# Autodesk Inventor assembly: ManualClamp
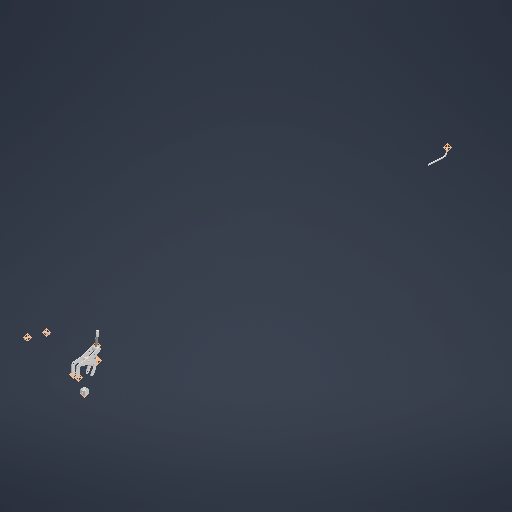
[picture p0: Inventor's stored thumbnail of the model, 512x512]
Saved by Autodesk Inventor 2025.4 (Build 294407000, 407)
## iProperties
Created: 2026-05-27
Part Number: ManualClamp
Document SubType Name: Assembly
Designer: VuQuan
Author: VuQuan
## Documents named in this file (12)
- D:\Edu\4CHaUI-Inventor\Assambly\b1\clamp\ManualClamp.iam
- D:\Edu\4CHaUI-Inventor\Assambly\b1\clamp\Base.ipt
- D:\Edu\4CHaUI-Inventor\Assambly\b1\clamp\BaseSpacer.ipt
- D:\Edu\4CHaUI-Inventor\Assambly\b1\clamp\BaseSupport.ipt
- D:\Edu\4CHaUI-Inventor\Assambly\b1\clamp\Elbow.ipt
- D:\Edu\4CHaUI-Inventor\Assambly\b1\clamp\Foot.ipt
- D:\Edu\4CHaUI-Inventor\Assambly\b1\clamp\FootPin.ipt
- D:\Edu\4CHaUI-Inventor\Assambly\b1\clamp\Hinge.ipt
- D:\Edu\4CHaUI-Inventor\Assambly\b1\clamp\Lever.ipt
- D:\Edu\4CHaUI-Inventor\Assambly\b1\clamp\Rod.ipt
- D:\Edu\4CHaUI-Inventor\Assambly\b1\clamp\Tee.ipt
- D:\Edu\4CHaUI-Inventor\Assambly\b1\clamp\Elbow_MIR.ipt
## Components (12 placed, 11 different names)
1. Base:1 — Insert:3, Insert:5, Mate:2
2. BaseSpacer:1 — Insert:5, Insert:6, Mate:4
3. BaseSupport:1
4. Elbow:1 — Insert:1, Insert:3, Mate:6
5. Foot:1
6. FootPin:1
7. Hinge:1 — Insert:1, Insert:2
8. Lever:1 — Mate:3
9. Rod:1 — Mate:3, Mate:4, Mate:5
10. Tee:1 — Mate:5, Mate:6, Mate:7
11. Base:2 — Insert:4, Insert:6
12. Elbow_MIR:1 — Insert:2, Insert:4, Mate:7
## Relationships (12: Insert 6, Mate 6)
- Insert:1: Elbow:1 ↔ Hinge:1
- Insert:2: Hinge:1 ↔ Elbow_MIR:1
- Insert:3: Base:1 ↔ Elbow:1
- Insert:4: Base:2 ↔ Elbow_MIR:1
- Insert:5: Base:1 ↔ BaseSpacer:1
- Insert:6: BaseSpacer:1 ↔ Base:2
- Mate:2: Base:1
- Mate:3: Lever:1 ↔ Rod:1
- Mate:4: BaseSpacer:1 ↔ Rod:1
- Mate:5: Rod:1 ↔ Tee:1
- Mate:6: Elbow:1 ↔ Tee:1
- Mate:7: Tee:1 ↔ Elbow_MIR:1
